# Autodesk Inventor assembly: MONTAGEM
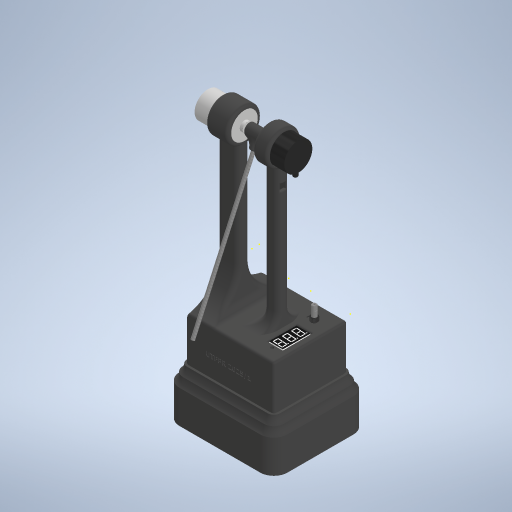
[picture p0: Inventor's stored thumbnail of the model, 512x512]
Saved by Autodesk Inventor 2024.1 (Build 281209000, 209)
## iProperties
Created: 2024-12-19
Part Number: MONTAGEM
Document SubType Name: Assembly
Designer: dimit
Author: dimit
## Documents named in this file (10)
- C:\Users\dimit\OneDrive\Área de Trabalho\3D\MONTAGEM.iam
- C:\Users\dimit\OneDrive\Área de Trabalho\Pendulo\Base.ipt
- C:\Users\dimit\Downloads\ROTARY ENCODER orange\ROTARY ENCODER orange.ipt
- C:\Users\dimit\OneDrive\Área de Trabalho\Pendulo\MOTOR.ipt
- C:\Users\dimit\OneDrive\Área de Trabalho\Pendulo\Montagem1\Design Accelerator\Engrenagens retas2.iam
- C:\Users\dimit\Downloads\DL7A-3 WHITE\DL7A-3 WHITE.ipt
- C:\Users\dimit\Downloads\EVQV9_RotaryEncoder\EVQV9_RotaryEncoder.ipt
- C:\Users\dimit\OneDrive\Área de Trabalho\Pendulo\acoplamento.ipt
- C:\Users\dimit\OneDrive\Área de Trabalho\Pendulo\BARRA.ipt
- C:\Users\dimit\OneDrive\Área de Trabalho\Pendulo\Peça1.ipt
## Components (9 placed, 9 different names)
1. Base:1 — Rotativa:1, Rotativa:2, Coincidente:1
2. ROTARY ENCODER orange:1 — Rotativa:1
3. MOTOR:1 — Rotativa:2, Rotativa:3
4. Engrenagens retas:1 [sub-assembly]
5. DL7A-3 WHITE:1
6. EVQV9_RotaryEncoder:1
7. acoplamento:1 — Rotativa:3, Rígida:1
8. BARRA:1 — Rígida:1
9. Peça1:1 — Coincidente:1
## Relationships (5: RevoluteJoint 3, WeldJoint 1, Mate 1)
- Rotativa:1 [RevoluteJoint]: Base:1 ↔ ROTARY ENCODER orange:1
- Rotativa:2 [RevoluteJoint]: Base:1 ↔ MOTOR:1
- Rotativa:3 [RevoluteJoint]: MOTOR:1 ↔ acoplamento:1
- Rígida:1 [WeldJoint]: acoplamento:1 ↔ BARRA:1
- Coincidente:1 [Mate]: Base:1 ↔ Peça1:1
